# Autodesk Inventor assembly: Assembly37
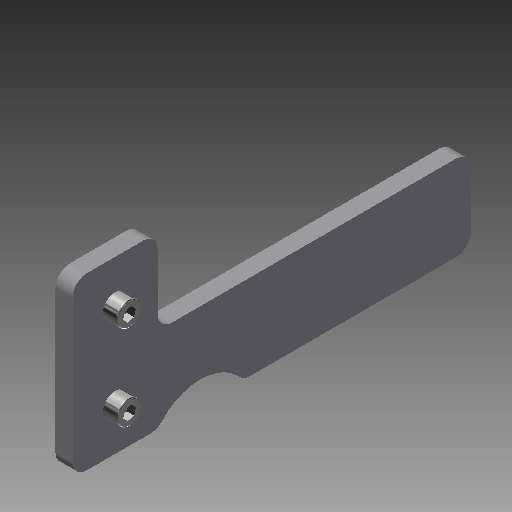
[picture p0: Inventor's stored thumbnail of the model, 512x512]
Saved by Autodesk Inventor 2017 (Build 210142000, 142)
## iProperties
Created: 2016-08-03
Part Number: Assembly37
Document SubType Name: Assembly
Designer: User
Author: User
## Documents named in this file (4)
- C:\All INVENTOR\SL-Inventor\SL-Beast 3D Printer\Assembly37.iam
- C:\All INVENTOR\SL-Inventor\SL-Beast 3D Printer\Spool Holder.ipt
- C:\All INVENTOR\SL-Inventor\SL-Beast 3D Printer\en-US\ANSI B18.3.1M(6)\ANSI B18.3.1M - M5x0.8 x 16(1).ipt
- C:\All INVENTOR\SL-Inventor\SL-Beast 3D Printer\M5 Tee Nut-Generic_MIR_CPY_MIR_MIR.ipt
## Components (5 placed, 3 different names)
1. Spool Holder:1
2. Forged Socket Head Cap Screw - Metric M5x0.8 x 16:1
3. Forged Socket Head Cap Screw - Metric M5x0.8 x 16:2
4. M5 Tee Nut-Generic_MIR_CPY_MIR_MIR:1
5. M5 Tee Nut-Generic_MIR_CPY_MIR_MIR:2
## Relationships (6: Mate 3, Insert 2, Flush 1)
- [Insert]: Spool Holder:1 ↔ Forged Socket Head Cap Screw - Metric M5x0.8 x 16:1
- [Insert]: Spool Holder:1 ↔ Forged Socket Head Cap Screw - Metric M5x0.8 x 16:2
- [Mate]: Forged Socket Head Cap Screw - Metric M5x0.8 x 16:1 ↔ M5 Tee Nut-Generic_MIR_CPY_MIR_MIR:1
- [Mate]: Forged Socket Head Cap Screw - Metric M5x0.8 x 16:2 ↔ M5 Tee Nut-Generic_MIR_CPY_MIR_MIR:2
- [Flush]: M5 Tee Nut-Generic_MIR_CPY_MIR_MIR:1 ↔ M5 Tee Nut-Generic_MIR_CPY_MIR_MIR:2
- [Mate] (6 mm): Spool Holder:1 ↔ M5 Tee Nut-Generic_MIR_CPY_MIR_MIR:1
